# Autodesk Inventor assembly: IBeam
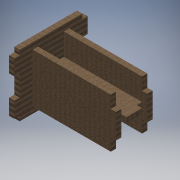
[picture p0: Inventor's stored thumbnail of the model, 180x180]
Saved by Autodesk Inventor 2016 (Build 200138000, 138)
## iProperties
Created: 2016-01-07
Part Number: IBeam
Document SubType Name: Assembly
Designer: m2memari
Author: m2memari
## Documents named in this file (4)
- C:\MoDonGD\Jane\ShadowGame\ShadowGame\IBeam.iam
- C:\MoDonGD\Jane\ShadowGame\ShadowGame\IBeamHorizantal.ipt
- C:\MoDonGD\Jane\ShadowGame\ShadowGame\IBeamVertical.ipt
- C:\MoDonGD\Jane\ShadowGame\ShadowGame\LightDiskSupport.ipt
## Components (4 placed, 3 different names)
1. IBeamHorizantal:1 — Mate:1, Mate:2, Mate:3, Mate:4, Mate:5, Mate:6, Mate:7
2. IBeamVertical:1 — Mate:1, Mate:2, Mate:3, Mate:8, Mate:9
3. LightDiskSupport:1 — Mate:7, Mate:8, Mate:9
4. IBeamVertical:2 — Mate:4, Mate:5, Mate:6
## Relationships (9: Mate 9)
- Mate:1: IBeamHorizantal:1 ↔ IBeamVertical:1
- Mate:2: IBeamHorizantal:1 ↔ IBeamVertical:1
- Mate:3: IBeamHorizantal:1 ↔ IBeamVertical:1
- Mate:4: IBeamHorizantal:1 ↔ IBeamVertical:2
- Mate:5: IBeamHorizantal:1 ↔ IBeamVertical:2
- Mate:6: IBeamHorizantal:1 ↔ IBeamVertical:2
- Mate:7: IBeamHorizantal:1 ↔ LightDiskSupport:1
- Mate:8: IBeamVertical:1 ↔ LightDiskSupport:1
- Mate:9: IBeamVertical:1 ↔ LightDiskSupport:1
